# Autodesk Inventor assembly: 組合1
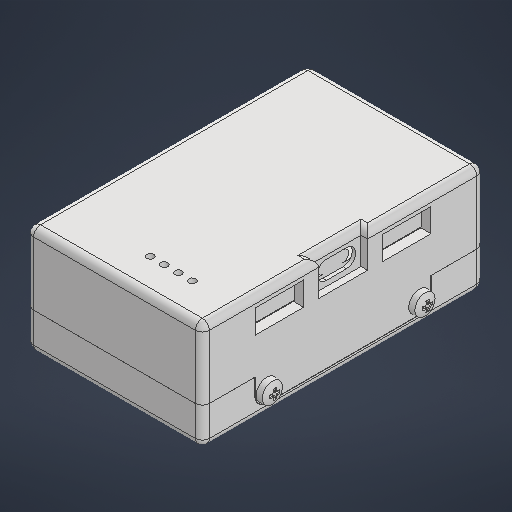
[picture p0: Inventor's stored thumbnail of the model, 512x512]
Saved by Autodesk Inventor 2026.3 (Build 303398000, 398)
## iProperties
Created: 2026-03-29
Part Number: 組合1
Document SubType Name: Assembly
Designer: gavin
Author: gavin
## Documents named in this file (7)
- D:\Inventor\power bank v1.1 mini\組合1.iam
- D:\Inventor\power bank v1.1 mini\18650 budge head.ipt
- D:\Inventor\power bank v1.1 mini\circuit board.ipt
- D:\Inventor\power bank v1.1 mini\buttom case.ipt
- D:\Inventor\power bank v1.1 mini\top case.ipt
- D:\Inventor\power bank v1.1 mini\botton.ipt
- D:\Inventor\power bank v1.1 mini\DIN 7985 (H) - M3x5-H.ipt
## Components (11 placed, 6 different names)
1. circuit board:1 — 貼合:5, 貼合:6, 剛性:5, 剛性:6
2. 18650 budge head:5 — 貼合:1, 相切:5, 貼合:2
3. buttom case:1 — 貼合:1, 相切:5, 貼合:2, 齊平:5, 齊平:6, 貼合:3
4. top case:1 — 齊平:5, 齊平:6, 貼合:3, 貼合:5, 貼合:6, 剛性:1, 剛性:2, 剛性:3, 剛性:4
5. botton:1
6. DIN 7985 (H) - M3x5-H:1 — 剛性:1
7. DIN 7985 (H) - M3x5-H:2 — 剛性:2
8. DIN 7985 (H) - M3x5-H:3 — 剛性:6
9. DIN 7985 (H) - M3x5-H:4 — 剛性:3
10. DIN 7985 (H) - M3x5-H:5 — 剛性:5
11. DIN 7985 (H) - M3x5-H:6 — 剛性:4
## Relationships (14: WeldJoint 6, Mate 5, Flush 2, Tangent 1)
- 貼合:1 [Mate]: 18650 budge head:5 ↔ buttom case:1
- 相切:5 [Tangent]: 18650 budge head:5 ↔ buttom case:1
- 貼合:2 [Mate]: 18650 budge head:5 ↔ buttom case:1
- 齊平:5 [Flush]: buttom case:1 ↔ top case:1
- 齊平:6 [Flush]: buttom case:1 ↔ top case:1
- 貼合:3 [Mate]: buttom case:1 ↔ top case:1
- 貼合:5 [Mate] (0.1 mm): circuit board:1 ↔ top case:1
- 貼合:6 [Mate] (0.38 mm): circuit board:1 ↔ top case:1
- 剛性:1 [WeldJoint]: top case:1 ↔ DIN 7985 (H) - M3x5-H:1
- 剛性:2 [WeldJoint]: top case:1 ↔ DIN 7985 (H) - M3x5-H:2
- 剛性:3 [WeldJoint]: top case:1 ↔ DIN 7985 (H) - M3x5-H:4
- 剛性:4 [WeldJoint]: top case:1 ↔ DIN 7985 (H) - M3x5-H:6
- 剛性:5 [WeldJoint]: circuit board:1 ↔ DIN 7985 (H) - M3x5-H:5
- 剛性:6 [WeldJoint]: circuit board:1 ↔ DIN 7985 (H) - M3x5-H:3
